# Autodesk Inventor assembly: TapeMeasureAssembly
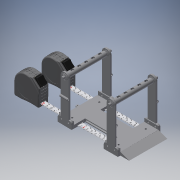
[picture p0: Inventor's stored thumbnail of the model, 180x180]
Saved by Autodesk Inventor 2019 (Build 230136000, 136)
## iProperties
Created: 2018-11-08
Part Number: TapeMeasureAssembly
Document SubType Name: Assembly
Designer: Ashley
Author: Ashley
## Documents named in this file (8)
- C:\Users\Ashley\Desktop\repositories\design\inventor\2018-2019\TapeMeasureAssembly.iam
- C:\Users\Ashley\Desktop\repositories\design\inventor\2018-2019\TapeMeasureBracketBottom.ipt
- C:\Users\Ashley\Desktop\repositories\design\inventor\2018-2019\Tape Measure Edited.iam
- C:\Users\Ashley\Desktop\repositories\design\inventor\2018-2019\TapeMeasureBracketTop.ipt
- C:\Users\Ashley\Desktop\repositories\design\inventor\2018-2019\TapeMeasureBracketSide.ipt
- C:\Users\Ashley\Desktop\repositories\design\inventor\Imported Components\goBilda\Bearing6mmID.ipt
- C:\Users\Ashley\Desktop\repositories\design\inventor\Imported Components\goBilda\DShaft120mm.ipt
- C:\Users\Ashley\Desktop\repositories\design\inventor\2018-2019\Spinner94mmDShaft.ipt
## Components (16 placed, 7 different names)
1. TapeMeasureBracketBottom:1 — Mate:1, Mate:2
2. Tape Measure Edited:1 [sub-assembly]
3. Tape Measure Edited:2 [sub-assembly]
4. TapeMeasureBracketTop:1
5. TapeMeasureBracketSide:1
6. TapeMeasureBracketSide:2 — Mate:1, Insert:2
7. TapeMeasureBracketSide:3 — Insert:3
8. TapeMeasureBracketSide:4 — Mate:2, Insert:4
9. Bearing6mmID:1 — Insert:8
10. Bearing6mmID:2 — Insert:2, Insert:7
11. Bearing6mmID:3 — Insert:3
12. Bearing6mmID:4 — Insert:4
13. DShaft120mm:2 — Insert:6, Insert:7
14. DShaft120mm:3 — Insert:5, Insert:8
15. Spinner94mmDShaft:1 — Insert:5
16. Spinner94mmDShaft:2 — Insert:6
## Relationships (9: Insert 7, Mate 2)
- Mate:1: TapeMeasureBracketBottom:1 ↔ TapeMeasureBracketSide:2
- Mate:2: TapeMeasureBracketBottom:1 ↔ TapeMeasureBracketSide:4
- Insert:2: TapeMeasureBracketSide:2 ↔ Bearing6mmID:2
- Insert:3: TapeMeasureBracketSide:3 ↔ Bearing6mmID:3
- Insert:4: TapeMeasureBracketSide:4 ↔ Bearing6mmID:4
- Insert:5 (13 mm): DShaft120mm:3 ↔ Spinner94mmDShaft:1
- Insert:6 (13 mm): DShaft120mm:2 ↔ Spinner94mmDShaft:2
- Insert:7 (5.5 mm): Bearing6mmID:2 ↔ DShaft120mm:2
- Insert:8 (5.5 mm): Bearing6mmID:1 ↔ DShaft120mm:3
